# Autodesk Inventor assembly: ATE2_Levas
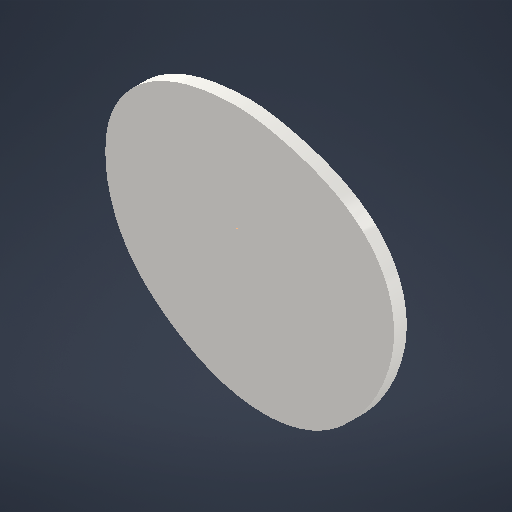
[picture p0: Inventor's stored thumbnail of the model, 512x512]
Saved by Autodesk Inventor 2026 (Build 300175050, 175E)
## iProperties
Created: 2025-12-05
Part Number: ATE2_Levas
Document SubType Name: Assembly
Designer: Usuario
Author: Usuario
## Documents named in this file (2)
- C:\Users\Usuario\Documents\ATE2_Levas.iam
- C:\Users\Usuario\Documents\Leva de disco1.ipt
## Components (1 placed, 1 different names)
1. Leva de disco:1 — Coincidencia:1
## Relationships (1: Mate 1)
- Coincidencia:1 [Mate]: Leva de disco:1
